# Autodesk Inventor assembly: Head
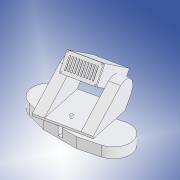
[picture p0: Inventor's stored thumbnail of the model, 180x180]
Saved by Autodesk Inventor 2017 (Build 210142000, 142)
## iProperties
Created: 2017-06-08
Part Number: Head
Document SubType Name: Assembly
Designer: zallen
Author: zallen
## Documents named in this file (8)
- C:\Users\zallen\Documents\GitHub\cr-laundry-robot\src\Head\Head.iam
- C:\Users\zallen\Documents\GitHub\cr-laundry-robot\src\Head\HA001.ipt
- C:\Users\zallen\Documents\GitHub\cr-laundry-robot\src\Head\HA002.ipt
- C:\Users\zallen\Documents\GitHub\cr-laundry-robot\src\Head\HA003.ipt
- C:\Users\zallen\Documents\GitHub\cr-laundry-robot\src\Head\HA004.ipt
- C:\Users\zallen\Documents\GitHub\cr-laundry-robot\src\Head\HA005.ipt
- C:\Users\zallen\Documents\GitHub\cr-laundry-robot\src\Head\HA006.ipt
- C:\Users\zallen\Documents\GitHub\cr-laundry-robot\lib\Stepper Motor - NEMA 17\NEMA17.ipt
## Components (7 placed, 7 different names)
1. HA001:1
2. HA002:1 — Mate:1, Mate:2, Mate:3, Mate:4, Mate:9, Mate:10, Mate:14
3. HA003:1 — Mate:2, Mate:3, Mate:4, Mate:5, Mate:6, Mate:15, Mate:16
4. HA004:1 — Mate:5, Mate:6, Mate:7, Mate:8
5. HA005:1 — Mate:7, Mate:8, Mate:11, Mate:12, Mate:13
6. HA006:1 — Mate:11, Mate:12, Mate:13
7. NEMA17:1 — Mate:14, Mate:15, Mate:16
## Relationships (16: Mate 16)
- Mate:1: HA002:1
- Mate:2: HA002:1 ↔ HA003:1
- Mate:3: HA002:1 ↔ HA003:1
- Mate:4: HA002:1 ↔ HA003:1
- Mate:5: HA003:1 ↔ HA004:1
- Mate:6: HA003:1 ↔ HA004:1
- Mate:7: HA004:1 ↔ HA005:1
- Mate:8: HA004:1 ↔ HA005:1
- Mate:9: HA002:1
- Mate:10: HA002:1
- Mate:11: HA005:1 ↔ HA006:1
- Mate:12: HA005:1 ↔ HA006:1
- Mate:13: HA005:1 ↔ HA006:1
- Mate:14: HA002:1 ↔ NEMA17:1
- Mate:15: HA003:1 ↔ NEMA17:1
- Mate:16: HA003:1 ↔ NEMA17:1
